# Autodesk Inventor assembly: Coluna_Suspensao_4-Cabos
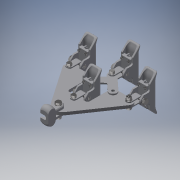
[picture p0: Inventor's stored thumbnail of the model, 180x180]
Saved by Autodesk Inventor 2018 (Build 220112000, 112)
## iProperties
Created: 2021-08-02
Part Number: Coluna_Suspensao_4-Cabos
Document SubType Name: Assembly
Designer: L08619
Author: L08619
## Documents named in this file (5)
- C:\Users\l08619\Documents\Projetos\TAESA\Modelo 3D - Tensionadores e Suspensão\Suporte de Suspenção\Coluna_Suspensao_4-Cabos.iam
- C:\Users\l08619\Documents\Projetos\TAESA\Modelo 3D - Tensionadores e Suspensão\Suporte de Suspenção\Corpo_Suporte_4_Cabos_Modelo3.ipt
- C:\Users\l08619\Documents\Projetos\TAESA\Modelo 3D - Tensionadores e Suspensão\Suporte de Suspenção\Suporte.ipt
- C:\Users\l08619\Documents\Projetos\TAESA\Modelo 3D - Tensionadores e Suspensão\Suporte de Suspenção\Clevis-Socket.iam
- C:\Users\l08619\Documents\Projetos\TAESA\Modelo 3D - Tensionadores e Suspensão\Suporte de Suspenção\Suspenssion_Clamp.iam
## Components (8 placed, 4 different names)
1. Corpo_Suporte_4_Cabos_Modelo3:1 — Mate:1, Mate:2, Rotational:1, Rotational:3, Mate:3, Cylindrical:1, Cylindrical:2, Cylindrical:3, Cylindrical:4, Mate:4, Mate:5, Mate:6, Mate:8
2. Suporte:1 — Rotational:1, Cylindrical:5, Mate:7
3. Suporte:4 — Rotational:3, Cylindrical:6
4. Clevis-Socket:1 [sub-assembly] — Cylindrical:1, Mate:4
5. Suspenssion_Clamp:1 [sub-assembly] — Cylindrical:2, Mate:5
6. Suspenssion_Clamp:2 [sub-assembly] — Cylindrical:3, Mate:6
7. Suspenssion_Clamp:3 [sub-assembly] — Cylindrical:4, Mate:8
8. Suspenssion_Clamp:4 [sub-assembly] — Cylindrical:5, Cylindrical:6, Mate:7
## Relationships (16: Mate 8, CylindricalJoint 6, RevoluteJoint 2)
- Mate:1: Corpo_Suporte_4_Cabos_Modelo3:1
- Mate:2: Corpo_Suporte_4_Cabos_Modelo3:1
- Rotational:1 [RevoluteJoint]: Corpo_Suporte_4_Cabos_Modelo3:1 ↔ Suporte:1
- Rotational:3 [RevoluteJoint]: Corpo_Suporte_4_Cabos_Modelo3:1 ↔ Suporte:4
- Mate:3: Corpo_Suporte_4_Cabos_Modelo3:1
- Cylindrical:1: Corpo_Suporte_4_Cabos_Modelo3:1 ↔ Clevis-Socket:1
- Cylindrical:2: Corpo_Suporte_4_Cabos_Modelo3:1 ↔ Suspenssion_Clamp:1
- Cylindrical:3: Corpo_Suporte_4_Cabos_Modelo3:1 ↔ Suspenssion_Clamp:2
- Cylindrical:4: Corpo_Suporte_4_Cabos_Modelo3:1 ↔ Suspenssion_Clamp:3
- Cylindrical:5: Suporte:1 ↔ Suspenssion_Clamp:4
- Cylindrical:6: Suporte:4 ↔ Suspenssion_Clamp:4
- Mate:4 (3 mm): Corpo_Suporte_4_Cabos_Modelo3:1 ↔ Clevis-Socket:1
- Mate:5 (3 mm): Corpo_Suporte_4_Cabos_Modelo3:1 ↔ Suspenssion_Clamp:1
- Mate:6 (3 mm): Corpo_Suporte_4_Cabos_Modelo3:1 ↔ Suspenssion_Clamp:2
- Mate:7 (6 mm): Suporte:1 ↔ Suspenssion_Clamp:4
- Mate:8 (3 mm): Corpo_Suporte_4_Cabos_Modelo3:1 ↔ Suspenssion_Clamp:3
